# Autodesk Inventor assembly: Assy
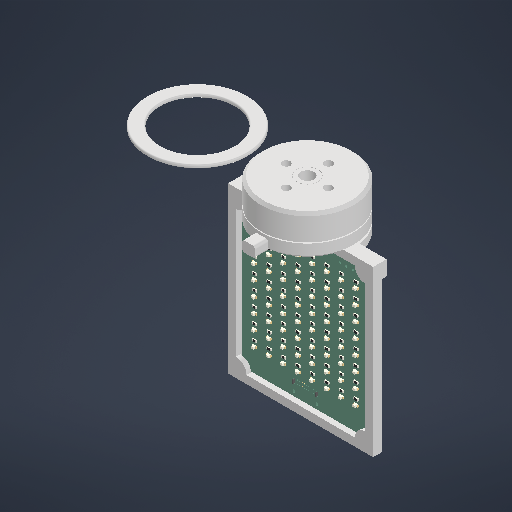
[picture p0: Inventor's stored thumbnail of the model, 512x512]
Saved by Autodesk Inventor 2026.1 (Build 301233020, 233B)
## iProperties
Created: 2026-09-21
Part Number: Assy
Document SubType Name: Assembly
Designer: InventorKid
Author: InventorKid
## Documents named in this file (5)
- D:\Projects\BYU_IEEE_2026_VOL_DISP\Holder\Assy.iam
- C:\Users\InventorKid\Downloads\VolumetricDisplay\VolumetricDisplay\VolumetricDisplay.iam
- D:\Projects\BYU_IEEE_2026_VOL_DISP\Holder\Frame.ipt
- D:\Projects\BYU_IEEE_2026_VOL_DISP\Rough Draft Cad\Motor.ipt
- D:\Projects\BYU_IEEE_2026_VOL_DISP\Rough Draft Cad\Coil.ipt
## Components (4 placed, 4 different names)
1. VolumetricDisplay:1 [sub-assembly] — Mate:2, Flush:1, Mate:3
2. Frame:1 — Mate:2, Flush:1, Mate:3, Insert:1, Insert:2
3. Motor:1 — Insert:1, Mate:4, Insert:2
4. Coil:1 — Mate:4
## Relationships (6: Mate 3, Insert 2, Flush 1)
- Mate:2 (0.15 mm): VolumetricDisplay:1 ↔ Frame:1
- Flush:1: VolumetricDisplay:1 ↔ Frame:1
- Mate:3 (0.15 mm): VolumetricDisplay:1 ↔ Frame:1
- Insert:1 (-1 mm): Frame:1 ↔ Motor:1
- Mate:4: Motor:1 ↔ Coil:1
- Insert:2 (-1 mm): Frame:1 ↔ Motor:1
